# Autodesk Inventor assembly: MAXPlanetary 3-Stage
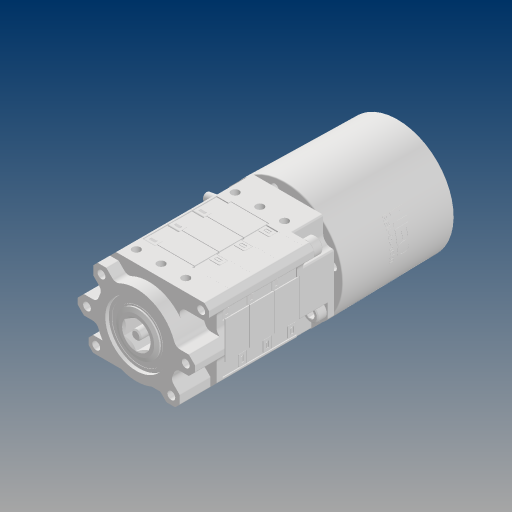
[picture p0: Inventor's stored thumbnail of the model, 512x512]
Saved by Autodesk Inventor 2024.3 (Build 283343000, 343)
## iProperties
Created: 2022-01-14
Part Number: MAXPlanetary 3-Stage
Description: STEP AP203
Document SubType Name: Assembly
Designer: Kenji
Sending System: SolidWorks 2022
Preprocessor: SwSTEP 2.0
Title: MAXPlanetary 3-Stage.STEP
Revision Number: ANY
## Documents named in this file (6)
- C:\Users\Kenji\Documents\FRC\Offseason 2024\DragBarLinkage3\MAXPlanetary 3-Stage.iam
- C:\Users\Kenji\Downloads\MAXPlanetary 3-Stage\MAXPlanetary 3-Stage\REV-25-2109_3-Stage (No Shaft, For NEO).iam
- C:\Users\Kenji\Downloads\MAXPlanetary 3-Stage\MAXPlanetary 3-Stage\REV-21-2101.ipt
- C:\Users\Kenji\Downloads\MAXPlanetary 3-Stage\MAXPlanetary 3-Stage\REV-21-2102.ipt
- C:\Users\Kenji\Downloads\MAXPlanetary 3-Stage\MAXPlanetary 3-Stage\REV-21-2103.ipt
- C:\Users\Kenji\Downloads\REV-21-1650-V1.1\REV-21-1650-V1.1\REV-21-1650-V1.1.ipt
## Components (5 placed, 5 different names)
1. REV-25-2109_3-Stage (No Shaft, For NEO)_1 [sub-assembly] — Mate:1, Mate:2, Mate:3
2. REV-21-2101_2
3. REV-21-2102_3
4. REV-21-2103_4
5. REV-21-1650-V1.1:1 — Mate:1, Mate:2, Mate:3
## Relationships (3: Mate 3)
- Mate:1: REV-25-2109_3-Stage (No Shaft, For NEO)_1 ↔ REV-21-1650-V1.1:1
- Mate:2: REV-25-2109_3-Stage (No Shaft, For NEO)_1 ↔ REV-21-1650-V1.1:1
- Mate:3: REV-25-2109_3-Stage (No Shaft, For NEO)_1 ↔ REV-21-1650-V1.1:1
